# Autodesk Inventor assembly: FrontBottomTube
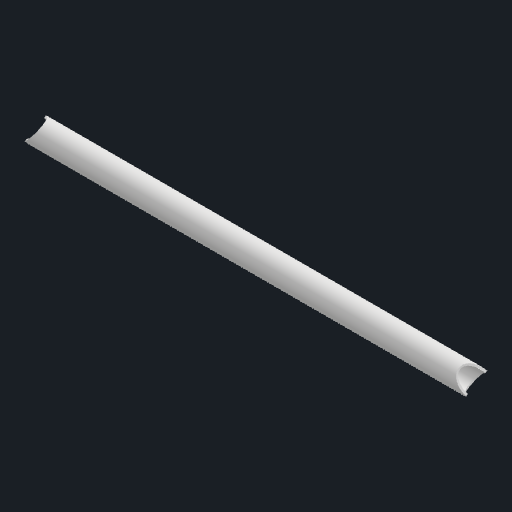
[picture p0: Inventor's stored thumbnail of the model, 512x512]
Saved by Autodesk Inventor 2025.2 (Build 292293000, 293)
## iProperties
Created: 2025-04-01
Part Number: FrontBottomTube
Document SubType Name: Assembly
Designer: valer
Author: valer
## Documents named in this file (2)
- C:\Users\valer\Desktop\str1ker\cad\FrontBottomTube.iam
- C:\Users\valer\Desktop\str1ker\cad\ChestFrontBottomTube.ipt
## Components (1 placed, 1 different names)
1. ChestFrontBottomTube:1 — Mate:1
## Relationships (1: Mate 1)
- Mate:1: ChestFrontBottomTube:1
